# Autodesk Inventor assembly: Assembly2
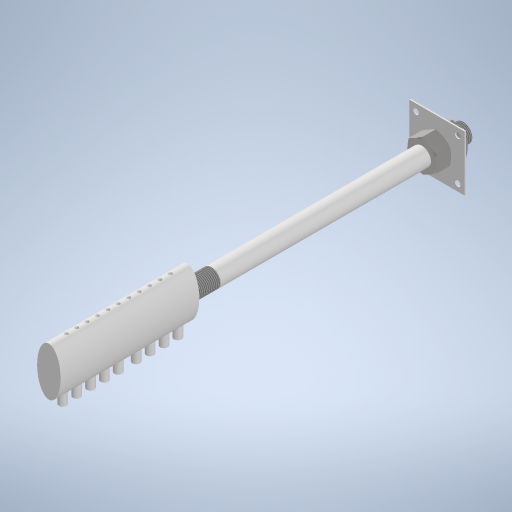
[picture p0: Inventor's stored thumbnail of the model, 512x512]
Saved by Autodesk Inventor 2023 (Build 270158000, 158)
## iProperties
Created: 2022-09-29
Part Number: Assembly2
Document SubType Name: Assembly
Designer: earls
Author: earls
## Documents named in this file (5)
- C:\Users\earls\Documents\stewart-platform\CAD\Smoke generator\Assembly2.iam
- C:\Users\earls\Documents\stewart-platform\CAD\Smoke generator\Threaded pipe.ipt
- C:\Users\earls\Documents\stewart-platform\CAD\Smoke generator\plate.ipt
- C:\Users\earls\Documents\stewart-platform\CAD\Smoke generator\Assembly1.iam
- C:\Users\earls\OneDrive\Documents\Inventor\Content Center Files\R2023\en-US\BS 3692(1)\BS 3692 - M27(1).ipt
## Components (5 placed, 4 different names)
1. Threaded pipe:1 — Mate:2, Mate:5, Rigid:1, Cylindrical:1, Mate:7
2. plate:1 — Mate:2, Mate:6, Mate:8
3. Assembly1:1 [sub-assembly] — Mate:5, Rigid:1
4. BS 3692 - Metric M27:1 — Cylindrical:1, Mate:6
5. BS 3692 - Metric M27:2 — Mate:7, Mate:8
## Relationships (7: Mate 5, WeldJoint 1, CylindricalJoint 1)
- Mate:2: Threaded pipe:1 ↔ plate:1
- Mate:5: Threaded pipe:1 ↔ Assembly1:1
- Rigid:1 [WeldJoint]: Threaded pipe:1 ↔ Assembly1:1
- Cylindrical:1: Threaded pipe:1 ↔ BS 3692 - Metric M27:1
- Mate:6: plate:1 ↔ BS 3692 - Metric M27:1
- Mate:7: Threaded pipe:1 ↔ BS 3692 - Metric M27:2
- Mate:8: plate:1 ↔ BS 3692 - Metric M27:2
